# Autodesk Inventor assembly: OpenFrame
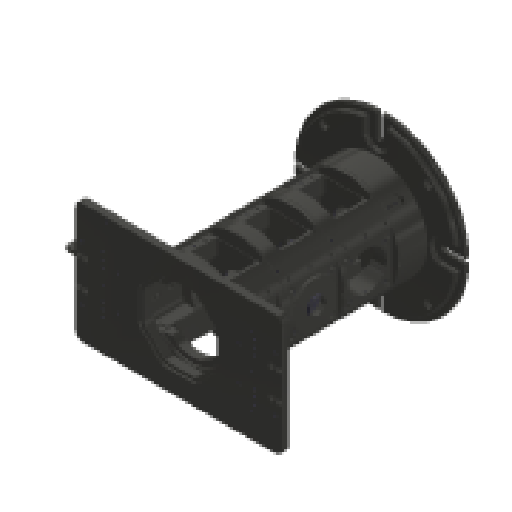
[picture p0: Inventor's stored thumbnail of the model, 512x512]
Saved by Autodesk Inventor 2024.1 (Build 281209000, 209)
## iProperties
Created: 2024-05-19
Part Number: OpenFrame
Document SubType Name: Assembly
Designer: AdminForWorker
Title: OpenFrame v1
Author: AdminForWorker
## Documents named in this file (10)
- C:\Users\diederichbenedict\Dropbox\Dokumente\Promotion\PROJECTS\SIMMO\INVENTOR\OpenFrame v1\OpenFrame.iam
- C:\Users\diederichbenedict\Dropbox\Dokumente\Promotion\PROJECTS\SIMMO\INVENTOR\OpenFrame v1\OF-LL-BP v1.ipt
- C:\Users\diederichbenedict\Dropbox\Dokumente\Promotion\PROJECTS\SIMMO\INVENTOR\OpenFrame v1\OpenFrame v1.iam
- C:\Users\diederichbenedict\Dropbox\Dokumente\Promotion\PROJECTS\SIMMO\INVENTOR\OpenFrame v1\OF-LL-FL-MOT v1.ipt
- C:\Users\diederichbenedict\Dropbox\Dokumente\Promotion\PROJECTS\SIMMO\INVENTOR\OpenFrame v1\OF-AD-SBSM2-CM v1.ipt
- C:\Users\diederichbenedict\Dropbox\Dokumente\Promotion\PROJECTS\SIMMO\INVENTOR\OpenFrame v1\OF-IN-MCH v1.ipt
- C:\Users\diederichbenedict\Dropbox\Dokumente\Promotion\PROJECTS\SIMMO\INVENTOR\OpenFrame v1\OF-LL-SP v1.ipt
- C:\Users\diederichbenedict\Dropbox\Dokumente\Promotion\PROJECTS\SIMMO\INVENTOR\00_openFrameExplodable5\OF-IN-MCH - cube _1__1_UC2_cube.iam
- C:\Users\diederichbenedict\Dropbox\Dokumente\Promotion\PROJECTS\SIMMO\INVENTOR\00_openFrameExplodable5\Assembly_Cube_empty_IM_v3\Assembly_Cube_empty_IM_v3.iam
- C:\Users\diederichbenedict\Dropbox\Dokumente\Promotion\PROJECTS\SIMMO\INVENTOR\OpenFrame v1\NAUO43_Tubelens_156.5_Astromedia.ipt
## Components (12 placed, 9 different names)
1. OpenFrame v1:1 [sub-assembly] — Einfügen:1
2. OF-LL-FL-MOT v1:1
3. OF-AD-SBSM2-CM v1:1
4. OF-IN-MCH v1:1
5. OF-LL-SP v1:1
6. OF-LL-BP v1:1 — Einfügen:2
7. OpenFrame v1:2 [sub-assembly] — Einfügen:1, Einfügen:2, Einfügen:3, Einfügen:4
8. OF-AD-SBSM2-CM v1:2 — Einfügen:3
9. OF-IN-MCH v1:2 — Einfügen:4
10. OF-IN-MCH - cube _1__1_UC2_cube:1 [sub-assembly]
11. Assembly_Cube_empty_IM_v3:1 [sub-assembly]
12. NAUO43_Tubelens_156.5_Astromedia:1
## Relationships (7: Insert 4, Mate 2, Angle 1)
- Einfügen:1 [Insert]: OpenFrame v1:1 ↔ OpenFrame v1:2
- Einfügen:2 [Insert]: OF-LL-BP v1:1 ↔ OpenFrame v1:2
- Einfügen:3 [Insert]: OpenFrame v1:2 ↔ OF-AD-SBSM2-CM v1:2
- Einfügen:4 [Insert] (-5 mm): OpenFrame v1:2 ↔ OF-IN-MCH v1:2
- [Mate]: OF-IN-MCH - cube _1__1_UC2_cube:1 ↔ Assembly_Cube_empty_IM_v3:1
- [Angle] (180 deg): OF-IN-MCH - cube _1__1_UC2_cube:1 ↔ Assembly_Cube_empty_IM_v3:1
- [Mate]: OF-IN-MCH - cube _1__1_UC2_cube:1 ↔ Assembly_Cube_empty_IM_v3:1
## Named parameters: d4_d0 = 0 mm, d5_d1 = 180 deg, d6_d2 = 0 mm
